# Autodesk Inventor assembly: Crankshaft Assembly
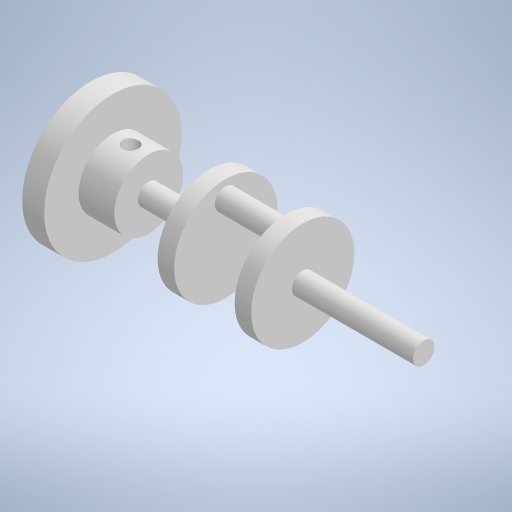
[picture p0: Inventor's stored thumbnail of the model, 512x512]
Saved by Autodesk Inventor 2023 (Build 270158000, 158)
## iProperties
Created: 2023-02-24
Part Number: Crankshaft Assembly
Document SubType Name: Assembly
Designer: tommy
Author: tommy
## Documents named in this file (5)
- C:\Users\tommy\Documents\Repositories\Steam-Engine\Les Proper Steam Engine\CAD\Crankshaft Assembly.iam
- C:\Users\tommy\Documents\Repositories\Steam-Engine\Les Proper Steam Engine\CAD\Flywheel.ipt
- C:\Users\tommy\Documents\Repositories\Steam-Engine\Les Proper Steam Engine\CAD\Crankshaft Crank Wheel.ipt
- C:\Users\tommy\Documents\Repositories\Steam-Engine\Les Proper Steam Engine\CAD\Crankshaft Crank.ipt
- C:\Users\tommy\Documents\Repositories\Steam-Engine\Les Proper Steam Engine\CAD\Crankshaft Engine Shaft.ipt
## Components (6 placed, 4 different names)
1. Flywheel:1 — Angle:2, Mate:5, Flush:5
2. Crankshaft Crank Wheel:1 — Mate:1, Angle:1, Angle:2, Flush:1, Flush:4, Mate:3
3. Crankshaft Crank:1 — Mate:1, Mate:2, Flush:1, Flush:2
4. Crankshaft Crank Wheel:2 — Mate:2, Angle:1, Flush:2, Flush:3, Mate:4
5. Crankshaft Engine Shaft:1 — Flush:4, Mate:3, Mate:5, Flush:5
6. Crankshaft Engine Shaft:2 — Flush:3, Mate:4
## Relationships (12: Mate 5, Flush 5, Angle 2)
- Mate:1: Crankshaft Crank Wheel:1 ↔ Crankshaft Crank:1
- Mate:2: Crankshaft Crank:1 ↔ Crankshaft Crank Wheel:2
- Angle:1 (0 deg): Crankshaft Crank Wheel:1 ↔ Crankshaft Crank Wheel:2
- Angle:2 (0 deg): Flywheel:1 ↔ Crankshaft Crank Wheel:1
- Flush:1: Crankshaft Crank Wheel:1 ↔ Crankshaft Crank:1
- Flush:2: Crankshaft Crank:1 ↔ Crankshaft Crank Wheel:2
- Flush:3: Crankshaft Crank Wheel:2 ↔ Crankshaft Engine Shaft:2
- Flush:4: Crankshaft Crank Wheel:1 ↔ Crankshaft Engine Shaft:1
- Mate:3: Crankshaft Crank Wheel:1 ↔ Crankshaft Engine Shaft:1
- Mate:4: Crankshaft Crank Wheel:2 ↔ Crankshaft Engine Shaft:2
- Mate:5: Flywheel:1 ↔ Crankshaft Engine Shaft:1
- Flush:5 (0.254 mm): Flywheel:1 ↔ Crankshaft Engine Shaft:1
